# Autodesk Inventor assembly: Kegelräder
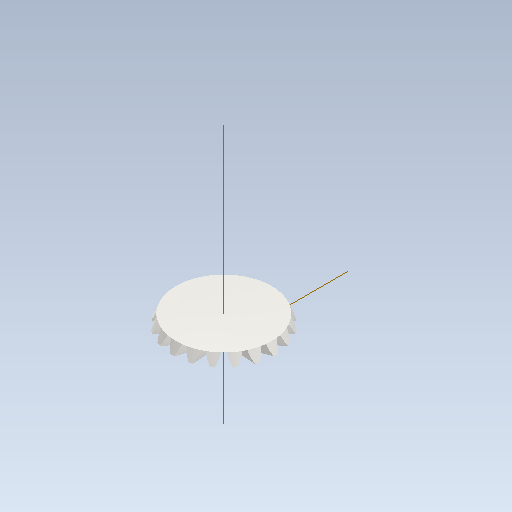
[picture p0: Inventor's stored thumbnail of the model, 512x512]
Saved by Autodesk Inventor 2021 (Build 250183000, 183)
## iProperties
ClientObjectVersion: 1
Created: 2021-01-23
Part Number: Kegelräder
Document SubType Name: Assembly
Designer: LETPJG
Categories: <?xml version="1.0" encoding="UTF-16"?> <MemberInstance><Categories><FamilyTemplate/><ParamToTemplateMap><ParamToTemplate><ParamToTemplate CategoryParameter="//CategoryParameter[@InternalName='9E91F9C2-1A37-4abf-91CE-B4CF7EE75BC6']" ConstantValue="10000000.000000"/></ParamToTemplate><ParamToTemplate><ParamToTemplate CategoryParameter="//CategoryParameter[@InternalName='2AFF4D85-1BD8-4ea8-8D18-96A2CAB0895B']" ConstantValue="9800000.000000"/></ParamToTemplate><ParamToTemplate><ParamToTemplate CategoryParameter="//CategoryParameter[@InternalName='E8E51088-10FD-40b5-B945-790B32C7EFBA']" ConstantValue="104.719755"/></ParamToTemplate><ParamToTemplate><ParamToTemplate CategoryParameter="//CategoryParameter[@InternalName='752D88A1-A866-440c-81C2-59259440B19C']" ConstantValue="41.887902"/></ParamToTemplate><ParamToTemplate><ParamToTemplate CategoryParameter="//CategoryParameter[@InternalName='5F43FD89-24D7-49f6-B63B-C3D8E39D8A69']" ConstantValue="95492.965855"/></ParamToTemplate><ParamToTemplate><ParamToTemplate CategoryParameter="//CategoryParameter[@InternalName='8D239626-6A17-497c-A9EF-C1C80B41D68F']" ConstantValue="233957.766345"/></ParamToTemplate><ParamToTemplate><ParamToTemplate CategoryParameter="//CategoryParameter[@InternalName='41D48E04-51D6-4192-AEE3-C42B8672B6EA']" ConstantValue="0.980000"/></ParamToTemplate><ParamToTemplate><ParamToTemplate CategoryParameter="//CategoryParameter[@InternalName='84837FB6-4F68-4020-B218-FAB91249D1CD']" ConstantValue="0.100000"/></ParamToTemplate><ParamToTemplate><ParamToTemplate CategoryParameter="//CategoryParameter[@InternalName='379FA8F8-BDC6-4dbf-8CB9-B54B76E22C20']" ConstantValue="10.000000"/></ParamToTemplate><ParamToTemplate><ParamToTemplate CategoryParameter="//CategoryParameter[@InternalName='2A36C5AF-6509-4e50-81F8-69CA9EC32B2C']" ConstantValue="0.349066"/></ParamToTemplate><ParamToTemplate><ParamToTemplate CategoryParameter="//CategoryParameter[@InternalName='E5FFB0D5-AABD-4279-8B19-7DCFF75B68C0']" ConstantValue="6"/></ParamToTemplate></ParamToTemplateMap><Category DisplayName="Gears" InternalName="3565AA18-AB10-415a-941E-C703DB507537" Mnemonic="Gears"><CategoryParameter DisplayName="P" InternalName="9E91F9C2-1A37-4abf-91CE-B4CF7EE75BC6" Mnemonic="P1"/><CategoryParameter DisplayName="P" InternalName="2AFF4D85-1BD8-4ea8-8D18-96A2CAB0895B" Mnemonic="P2"/><CategoryParameter DisplayName="n" InternalName="E8E51088-10FD-40b5-B945-790B32C7EFBA" Mnemonic="n1"/><CategoryParameter DisplayName="n" InternalName="752D88A1-A866-440c-81C2-59259440B19C" Mnemonic="n2"/><CategoryParameter DisplayName="T" InternalName="5F43FD89-24D7-49f6-B63B-C3D8E39D8A69" Mnemonic="Mk1"/><CategoryParameter DisplayName="T" InternalName="8D239626-6A17-497c-A9EF-C1C80B41D68F" Mnemonic="Mk2"/><CategoryParameter DisplayName="||h|" InternalName="41D48E04-51D6-4192-AEE3-C42B8672B6EA" Mnemonic="eta"/><Category DisplayName="BevelGears" InternalName="3F761496-A216-438c-BEB6-B38CAC295276" Mnemonic="BevelGears"><CategoryParameter DisplayName="m|.et|" InternalName="84837FB6-4F68-4020-B218-FAB91249D1CD" Mnemonic="met"/><CategoryParameter DisplayName="P|.et|" InternalName="379FA8F8-BDC6-4dbf-8CB9-B54B76E22C20" Mnemonic="Pet"/><CategoryParameter DisplayName="||a||.t|" InternalName="2A36C5AF-6509-4e50-81F8-69CA9EC32B2C" Mnemonic="alphat"/><CategoryParameter DisplayName="idxIT1" InternalName="E5FFB0D5-AABD-4279-8B19-7DCFF75B68C0" Mnemonic="idxIT1"/></Category></Category></Categories></MemberInstance>
Author: LETPJG
## Documents named in this file (3)
- C:\Users\LETPJG\Documents\Inventor\zahnstange\Planeten\Konstruktions-Assistent\Kegelräder10.iam
- C:\Users\LETPJG\Documents\Inventor\zahnstange\Planeten\Konstruktions-Assistent\Kegelrad110.ipt
- C:\Users\LETPJG\Documents\Inventor\zahnstange\Planeten\Konstruktions-Assistent\Kegelrad29.ipt
## Components (2 placed, 2 different names)
1. Kegelrad1:1 — Passend:1, Winkel:1, Drehung:1
2. Kegelrad2:1 — Passend:1, Winkel:1, Drehung:1
## Relationships (3: Mate 1, Angle 1, RelateRotation 1)
- Passend:1 [Mate]: Kegelrad1:1 ↔ Kegelrad2:1
- Winkel:1 [Angle] (90 deg): Kegelrad1:1 ↔ Kegelrad2:1
- Drehung:1 [RelateRotation] (0.4 ul): Kegelrad1:1 ↔ Kegelrad2:1
